# Autodesk Inventor assembly: brazo robot
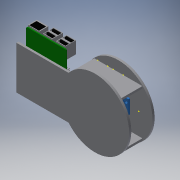
[picture p0: Inventor's stored thumbnail of the model, 180x180]
Saved by Autodesk Inventor 2018 (Build 220112000, 112)
## iProperties
Created: 2020-03-10
Part Number: brazo robot
Material: Genérico
Document SubType Name: Assembly
Designer: sala.ceri
Author: sala.ceri
## Documents named in this file (7)
- C:\Users\david\OneDrive\Documents\robot\ensamble\part1.iam
- C:\Users\david\OneDrive\Documents\robot\piezas\ServoMotor.ipt
- C:\Users\david\OneDrive\Documents\robot\piezas\BaseServo.ipt
- C:\Users\david\OneDrive\Documents\robot\base2.ipt
- C:\Users\david\OneDrive\Documents\robot\base3.ipt
- C:\Users\david\OneDrive\Documents\robot\base4.ipt
- C:\Users\david\OneDrive\Documents\robot\piezas\raspberry.ipt
## Components (7 placed, 6 different names)
1. base2:1 — Coincidencia:96, Coincidencia:97, Coincidencia:102, Coincidencia:103, Coincidencia:104, Coincidencia:105
2. ServoMotor:5 — Coincidencia:96, Coincidencia:97, Coincidencia:98, Coincidencia:99, Coincidencia:109
3. BaseServo:5 — Coincidencia:98, Coincidencia:99
4. base3:1 — Coincidencia:106, Coincidencia:107, Nivelación:6, Nivelación:7
5. base4:1 — Coincidencia:102, Coincidencia:103
6. base4:2 — Coincidencia:104, Coincidencia:105, Coincidencia:106, Coincidencia:107
7. raspberry:1 — Nivelación:6, Coincidencia:109, Nivelación:7
## Relationships (13: Mate 11, Flush 2)
- Coincidencia:96 [Mate]: base2:1 ↔ ServoMotor:5
- Coincidencia:97 [Mate]: base2:1 ↔ ServoMotor:5
- Coincidencia:98 [Mate]: ServoMotor:5 ↔ BaseServo:5
- Coincidencia:99 [Mate]: ServoMotor:5 ↔ BaseServo:5
- Coincidencia:102 [Mate]: base2:1 ↔ base4:1
- Coincidencia:103 [Mate]: base2:1 ↔ base4:1
- Coincidencia:104 [Mate]: base2:1 ↔ base4:2
- Coincidencia:105 [Mate]: base2:1 ↔ base4:2
- Coincidencia:106 [Mate]: base3:1 ↔ base4:2
- Coincidencia:107 [Mate]: base3:1 ↔ base4:2
- Nivelación:6 [Flush]: base3:1 ↔ raspberry:1
- Coincidencia:109 [Mate]: ServoMotor:5 ↔ raspberry:1
- Nivelación:7 [Flush]: base3:1 ↔ raspberry:1
